# Autodesk Inventor assembly: LowerBackLink
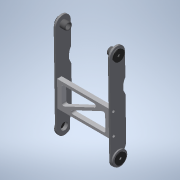
[picture p0: Inventor's stored thumbnail of the model, 180x180]
Saved by Autodesk Inventor 2020.4 (Build 244396000, 396)
## iProperties
Created: 2016-08-23
Part Number: LowerBackLink
Material: 一般
Document SubType Name: Assembly
Designer: hiro
Mass: 27.0677 g
Surface Area: 148.123 cm^2
Volume: 12.1706 cm^3
Density: 2.22402 g/cm^3
Author: hiro
## Documents named in this file (6)
- C:\Users\Masato\Documents\Inventor\CIT Brains_Inventor\OpenPlatform_ver3_0\下半身\リンク\LowerBackLink.iam
- C:\Users\Masato\Documents\Inventor\CIT Brains_Inventor\OpenPlatform_ver3_0\下半身\リンク\リンク_メインフレーム_6_1.ipt
- C:\Users\Masato\Documents\Inventor\CIT Brains_Inventor\OpenPlatform_ver3_0\下半身\リンク\リンク_ふくらはぎ_サブフレーム_1_2.ipt
- C:\Users\Masato\Documents\Inventor\CIT Brains_Inventor\OpenPlatform_ver3_0\Ready_Made\80F-0608.ipt
- C:\Users\Masato\Documents\Inventor\CIT Brains_Inventor\OpenPlatform_ver3_0\Ready_Made\UUW-0312-10BH.ipt
- C:\Users\Masato\Documents\Inventor\CIT Brains_Inventor\OpenPlatform_ver3_0\Ready_Made\LFW-0815.ipt
## Components (11 placed, 5 different names)
1. リンク_メインフレーム_6_1:1 — 挿入:14, 挿入:17, 挿入:21, 挿入:22
2. リンク_メインフレーム_6_1:2 — 挿入:13, 挿入:18, 挿入:23, 挿入:24
3. 80F-0608:1 — 挿入:13, 挿入:16
4. 80F-0608:2 — 挿入:14, 挿入:15
5. UUW-0312-10BH:1 — 挿入:15
6. UUW-0312-10BH:2 — 挿入:16
7. UUW-0312-10BH:3 — 挿入:20
8. UUW-0312-10BH:4 — 挿入:19
9. LFW-0815:1 — 挿入:18, 挿入:20
10. LFW-0815:2 — 挿入:17, 挿入:19
11. リンク_ふくらはぎ_サブフレーム_1_2:1 — 挿入:21, 挿入:22, 挿入:23, 挿入:24
## Relationships (12: Insert 12)
- 挿入:13 [Insert]: リンク_メインフレーム_6_1:2 ↔ 80F-0608:1
- 挿入:14 [Insert]: リンク_メインフレーム_6_1:1 ↔ 80F-0608:2
- 挿入:15 [Insert]: 80F-0608:2 ↔ UUW-0312-10BH:1
- 挿入:16 [Insert]: 80F-0608:1 ↔ UUW-0312-10BH:2
- 挿入:17 [Insert]: リンク_メインフレーム_6_1:1 ↔ LFW-0815:2
- 挿入:18 [Insert]: リンク_メインフレーム_6_1:2 ↔ LFW-0815:1
- 挿入:19 [Insert]: UUW-0312-10BH:4 ↔ LFW-0815:2
- 挿入:20 [Insert]: UUW-0312-10BH:3 ↔ LFW-0815:1
- 挿入:21 [Insert]: リンク_メインフレーム_6_1:1 ↔ リンク_ふくらはぎ_サブフレーム_1_2:1
- 挿入:22 [Insert]: リンク_メインフレーム_6_1:1 ↔ リンク_ふくらはぎ_サブフレーム_1_2:1
- 挿入:23 [Insert]: リンク_メインフレーム_6_1:2 ↔ リンク_ふくらはぎ_サブフレーム_1_2:1
- 挿入:24 [Insert]: リンク_メインフレーム_6_1:2 ↔ リンク_ふくらはぎ_サブフレーム_1_2:1
